# Autodesk Inventor assembly: Rack_Pinion
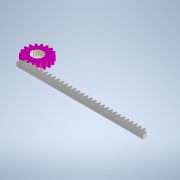
[picture p0: Inventor's stored thumbnail of the model, 180x180]
Saved by Autodesk Inventor 2022 (Build 260153000, 153)
## iProperties
Created: 2022-01-08
Part Number: Rack_Pinion
Document SubType Name: Assembly
Designer: Elia
Author: Elia
## Documents named in this file (3)
- C:\Users\Elia\Documents\UNITN\MAGISTRALE\1st year\1st semester\Mechanical Design\Project\MDM-CyberOrto-CAD-main\Rack_Pinion.iam
- C:\Users\Elia\Documents\UNITN\MAGISTRALE\1st year\1st semester\Mechanical Design\Project\MDM-CyberOrto-CAD-main\Pinion m10 Z18.ipt
- C:\Users\Elia\Documents\UNITN\MAGISTRALE\1st year\1st semester\Mechanical Design\Project\MDM-CyberOrto-CAD-main\Rack gear m10 Z30.ipt
## Components (2 placed, 2 different names)
1. Pinion m10 Z18:1 — Coincidente:1, Coincidente:2, Allineato:1, Coincidente:3, Tangente:1, Rotazione/Traslazione:1, Angolo:2
2. Rack gear m10 Z30:1 — Allineato:1, Coincidente:3, Angolo:1, Tangente:1, Rotazione/Traslazione:1, Angolo:2
## Relationships (8: Mate 3, Angle 2, Flush 1, Tangent 1, RelateRotateTranslate 1)
- Coincidente:1 [Mate]: Pinion m10 Z18:1
- Coincidente:2 [Mate]: Pinion m10 Z18:1
- Allineato:1 [Flush]: Pinion m10 Z18:1 ↔ Rack gear m10 Z30:1
- Coincidente:3 [Mate]: Pinion m10 Z18:1 ↔ Rack gear m10 Z30:1
- Angolo:1 [Angle] (180 deg): Rack gear m10 Z30:1
- Tangente:1: Pinion m10 Z18:1 ↔ Rack gear m10 Z30:1
- Rotazione/Traslazione:1 [RelateRotateTranslate] (565.4867 mm): Pinion m10 Z18:1 ↔ Rack gear m10 Z30:1
- Angolo:2 [Angle] (90 deg): Pinion m10 Z18:1 ↔ Rack gear m10 Z30:1
